# Autodesk Inventor assembly: AM14U3 Long Half
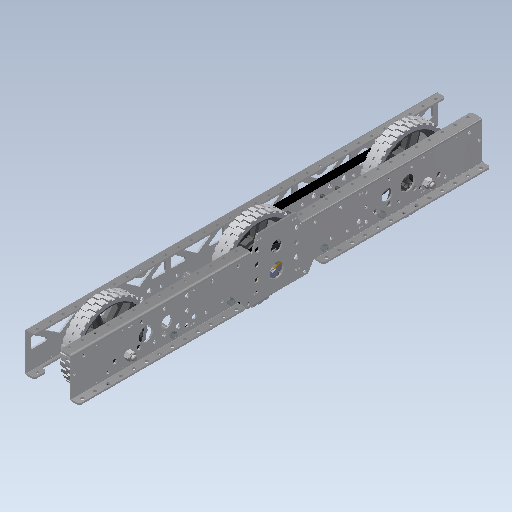
[picture p0: Inventor's stored thumbnail of the model, 512x512]
Saved by Autodesk Inventor 2020 (Build 240168000, 168)
## iProperties
Created: 2015-12-05
Part Number: AM14U3 Long Half
Document SubType Name: Assembly
Designer: PhillipD
Author: PhillipD
Revision Number: ANY
## Documents named in this file (8)
- C:\Users\srini\Documents\FRC\2020\2018_KOP\Inventor\FRC 2018 Drive Base Inventor\FIRST 2018 Drive Base\Parts\AM14U3 Long Half.iam
- C:\Users\srini\Documents\FRC\2020\2018_KOP\Inventor\FRC 2018 Drive Base Inventor\FIRST 2018 Drive Base\Parts\AM14U3 Long Frame Half.iam
- C:\Users\srini\Documents\FRC\2020\2018_KOP\Inventor\FRC 2018 Drive Base Inventor\FIRST 2018 Drive Base\Parts\6 HiGrip with bearings, pulleys and spacers.iam
- C:\Users\srini\Documents\FRC\2020\2018_KOP\Inventor\FRC 2018 Drive Base Inventor\FIRST 2018 Drive Base\Parts\6 HiGrip with hub and double pulley.iam
- C:\Users\srini\Documents\FRC\2020\2018_KOP\Inventor\FRC 2018 Drive Base Inventor\FIRST 2018 Drive Base\Parts\FR8ZZ Hex Bearing.ipt
- C:\Users\srini\Documents\FRC\2020\2018_KOP\Inventor\FRC 2018 Drive Base Inventor\FIRST 2018 Drive Base\Parts\am-2266 800-5M-15 v2 Timing Belt.ipt
- C:\Users\srini\Documents\FRC\2020\2018_KOP\Inventor\FRC 2018 Drive Base Inventor\FIRST 2018 Drive Base\Parts\375-16 x 4.25 Hex Bolt_HFBOLT 0.375-16x2.5x1-C.ipt
- C:\Users\srini\Documents\FRC\2020\2018_KOP\Inventor\FRC 2018 Drive Base Inventor\FIRST 2018 Drive Base\Parts\375-16 Lock Nut_91831A127.ipt
## Components (11 placed, 11 different names)
1. AM14U3 Long Frame Half_3 [sub-assembly] — Insert:1, Angle:1, Insert:2, Angle:2, Insert:3, Insert:4, Angle:3, Insert:5, Insert:6, Insert:7
2. 6 HiGrip with bearings, pulleys and spacers_4 [sub-assembly] — Insert:3
3. 6 HiGrip with bearings, pulleys and spacers_5 [sub-assembly] — Insert:6
4. 6 HiGrip with hub and double pulley_6 [sub-assembly] — Insert:8, Angle:4, Mate:1
5. FR8ZZ Hex Bearing_8 — Insert:7, Insert:8, Angle:4
6. am-2266 800-5M-15 v2 Timing Belt_9 — Mate:2
7. am-2266 800-5M-15 v2 Timing Belt_10 — Mate:1
8. 375-16 x 4.25 Hex Bolt_HFBOLT 0.375-16x2.5x1-C_11 — Insert:1, Angle:1, Mate:2
9. 375-16 x 4.25 Hex Bolt_HFBOLT 0.375-16x2.5x1-C_12 — Insert:4, Angle:3
10. 375-16 Lock Nut_91831A127_13 — Insert:5
11. 375-16 Lock Nut_91831A127_14 — Insert:2, Angle:2
## Relationships (14: Insert 8, Angle 4, Mate 2)
- Insert:1: AM14U3 Long Frame Half_3 ↔ 375-16 x 4.25 Hex Bolt_HFBOLT 0.375-16x2.5x1-C_11
- Angle:1 (0 deg): AM14U3 Long Frame Half_3 ↔ 375-16 x 4.25 Hex Bolt_HFBOLT 0.375-16x2.5x1-C_11
- Insert:2: AM14U3 Long Frame Half_3 ↔ 375-16 Lock Nut_91831A127_14
- Angle:2 (0 deg): AM14U3 Long Frame Half_3 ↔ 375-16 Lock Nut_91831A127_14
- Insert:3 (0.0762 mm): AM14U3 Long Frame Half_3 ↔ 6 HiGrip with bearings, pulleys and spacers_4
- Insert:4: AM14U3 Long Frame Half_3 ↔ 375-16 x 4.25 Hex Bolt_HFBOLT 0.375-16x2.5x1-C_12
- Angle:3 (0 deg): AM14U3 Long Frame Half_3 ↔ 375-16 x 4.25 Hex Bolt_HFBOLT 0.375-16x2.5x1-C_12
- Insert:5: AM14U3 Long Frame Half_3 ↔ 375-16 Lock Nut_91831A127_13
- Insert:6 (0.0762 mm): AM14U3 Long Frame Half_3 ↔ 6 HiGrip with bearings, pulleys and spacers_5
- Insert:7: AM14U3 Long Frame Half_3 ↔ FR8ZZ Hex Bearing_8
- Insert:8: 6 HiGrip with hub and double pulley_6 ↔ FR8ZZ Hex Bearing_8
- Angle:4 (10 deg): 6 HiGrip with hub and double pulley_6 ↔ FR8ZZ Hex Bearing_8
- Mate:1: 6 HiGrip with hub and double pulley_6 ↔ am-2266 800-5M-15 v2 Timing Belt_10
- Mate:2: am-2266 800-5M-15 v2 Timing Belt_9 ↔ 375-16 x 4.25 Hex Bolt_HFBOLT 0.375-16x2.5x1-C_11
